# Autodesk Inventor assembly: robot
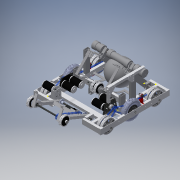
[picture p0: Inventor's stored thumbnail of the model, 180x180]
Saved by Autodesk Inventor 2016 (Build 200138000, 138)
## iProperties
Created: 2016-01-18
Part Number: robot
Document SubType Name: Assembly
Designer: gus
Mass: 30875.5 g
Surface Area: 55089.9 cm^2
Volume: 19218.2 cm^3
Density: 1.60657 g/cm^3
Author: gus
## Documents named in this file (36)
- \\Mac\Home\Desktop\1510-stronghold-CAD-master\robot.iam
- \\Mac\Home\Desktop\1510-stronghold-CAD-master\chassis\chassis.iam
- \\Mac\Home\Desktop\1510-stronghold-CAD-master\roller wheels\roller wheels.iam
- \\Mac\Home\Desktop\1510-stronghold-CAD-master\chassis\chain tensioner\chain tensioner.iam
- \\Mac\Home\Desktop\1510-stronghold-CAD-master\pickeruperthingy\armAssembaly.iam
- \\Mac\Home\Desktop\1510-stronghold-CAD-master\pickeruperthingy\2x2block.ipt
- \\Mac\Home\Desktop\1510-stronghold-CAD-master\pickeruperthingy\Roller Drum 10-Inch.ipt
- \\Mac\Home\Desktop\1510-stronghold-CAD-master\pickeruperthingy\Roller Drum 4-Inch.ipt
- \\Mac\Home\Desktop\1510-stronghold-CAD-master\roller wheels\4-in higrip\4 in HiGrip Wheel.iam
- \\Mac\Home\Desktop\1510-stronghold-CAD-master\pickeruperthingy\Part13.ipt
- \\Mac\Home\Desktop\1510-stronghold-CAD-master\shooter\Part4.ipt
- \\Mac\Home\Desktop\1510-stronghold-CAD-master\shooter\railtop.ipt
- \\Mac\Home\Desktop\1510-stronghold-CAD-master\shooter\superstructure.ipt
- \\Mac\Home\Desktop\1510-stronghold-CAD-master\shooter\supportbeam1.ipt
- \\Mac\Home\Desktop\1510-stronghold-CAD-master\shooter\supportblock1.ipt
- \\Mac\Home\Desktop\1510-stronghold-CAD-master\shooter\supportbeam2.ipt
- \\Mac\Home\Desktop\1510-stronghold-CAD-master\shooter\superstructure2.ipt
- \\Mac\Home\Desktop\1510-stronghold-CAD-master\shooter\flywheelsupport.ipt
- \\Mac\Home\Desktop\1510-stronghold-CAD-master\shooter\flywheelsupport2.ipt
- \\Mac\Home\Desktop\1510-stronghold-CAD-master\shooter\aimingrails.ipt
- \\Mac\Home\Desktop\1510-stronghold-CAD-master\shooter\bolt.ipt
- \\Mac\Home\Desktop\1510-stronghold-CAD-master\shooter\boltholder.ipt
- \\Mac\Home\Desktop\1510-stronghold-CAD-master\shooter\aimingcontrol.ipt
- \\Mac\Home\Desktop\1510-stronghold-CAD-master\pickeruperthingy\rollerwheelpoweraxel.ipt
- \\Mac\Home\Desktop\1510-stronghold-CAD-master\pickeruperthingy\217-3875-STEP-20140818.ipt
- \\Mac\Home\Desktop\1510-stronghold-CAD-master\roller wheels\am-0096a+500+Hex+Hub+r2.ipt
- \\Mac\Home\Desktop\1510-stronghold-CAD-master\pickeruperthingy\rod3.ipt
- \\Mac\Home\Desktop\1510-stronghold-CAD-master\pickeruperthingy\217-2704.20121204.ipt
- \\Mac\Home\Desktop\1510-stronghold-CAD-master\roller cage\roller cage.iam
- \\Mac\Home\Desktop\1510-stronghold-CAD-master\ball.ipt
- \\Mac\Home\Desktop\1510-stronghold-CAD-master\shooter\am-2231a+375+Hex+Hub+r3.ipt
- \\Mac\Home\Desktop\1510-stronghold-CAD-master\shooter\217-2735.20121205-2.ipt
- \\Mac\Home\Desktop\1510-stronghold-CAD-master\roller cage\3-8 hex axle.ipt
- \\Mac\Home\Desktop\1510-stronghold-CAD-master\shooter\fly wheel gusset.ipt
- \\Mac\Home\Desktop\1510-stronghold-CAD-master\shooter\angle gusset.ipt
- \\Mac\Home\Desktop\1510-stronghold-CAD-master\shooter\angle gusset 2.ipt
## Components (72 placed, 35 different names)
1. chassis:1 [sub-assembly] — Cylindrical:1, Mate:1, Flush:1, Mate:3, Flush:2, Mate:4, Mate:5, Flush:3, Flush:4, Flush:5, Flush:6, Mate:6, Mate:16, Flush:22, Mate:23, Flush:23, Flush:24, Mate:24, Mate:25, Mate:35, Mate:37, Mate:40, Mate:41, Flush:37, Mate:43, Flush:41, Mate:107, Mate:115, Flush:81, Flush:82, Mate:116, Flush:83, Mate:119
2. roller wheels:1 [sub-assembly] — Cylindrical:1, Mate:1
3. chain tensioner:1 [sub-assembly] — Flush:1
4. chain tensioner:2 [sub-assembly] — Mate:3, Flush:2
5. armAssembaly:1 [sub-assembly] — Mate:4, Mate:7, Mate:8, Mate:9, Mate:10, Mate:11, Mate:12, Flush:7, Mate:13, Mate:14, Flush:8, Flush:12, Flush:74, Mate:78, Mate:79, Mate:80, Mate:81
6. 2x2block:1 — Mate:5, Flush:3, Flush:4, Mate:76, Mate:77
7. 2x2block:2 — Flush:5, Flush:6, Mate:6, Mate:7, Mate:72, Mate:73
8. Roller Drum 10-Inch:1 — Mate:8, Mate:9, Mate:10, Mate:78
9. Roller Drum 4-Inch:1 — Mate:13, Mate:14, Flush:8
10. Roller Drum 4-Inch:2 — Mate:11, Mate:12, Flush:7
11. 4 in HiGrip Wheel:1 [sub-assembly] — Mate:47, Mate:88, Mate:89, Mate:90, Mate:91, Mate:92, Mate:93, Mate:107
12. Part13:1 — Mate:16, Flush:12, Mate:17, Flush:13, Flush:14, Mate:18, Flush:15, Mate:19, Mate:33, Flush:32, Mate:34
13. Part13:2 — Mate:17, Flush:13, Flush:14, Mate:25, Flush:33, Mate:36
14. Part4:1 — Mate:18, Flush:15, Mate:19, Mate:20, Flush:16, Flush:17, Flush:35, Flush:36, Mate:38, Flush:62, Mate:58, Flush:63, Flush:64
15. Part4:2 — Mate:20, Flush:16, Flush:17, Flush:18, Flush:19, Mate:21, Flush:39, Flush:40, Flush:58, Flush:59, Flush:60, Mate:56, Flush:61, Flush:66
16. railtop:1 — Flush:18, Flush:19, Mate:21, Mate:22, Flush:20, Flush:21, Flush:26, Flush:27, Flush:48, Flush:50
17. railtop:2 — Mate:22, Flush:20, Flush:21, Flush:29, Flush:30, Mate:53, Flush:53, Flush:54, Flush:55
18. superstructure:1 — Flush:22, Mate:23, Flush:23, Flush:25, Mate:29, Mate:31, Flush:34, Mate:39, Mate:40, Mate:87, Flush:76
19. superstructure:2 — Flush:24, Mate:24, Flush:25, Mate:26, Mate:28
20. supportbeam1:1 — Mate:26, Flush:26, Flush:27, Mate:27, Flush:28, Mate:49, Flush:51
21. supportblock1:1 — Mate:27, Flush:28, Mate:28
22. supportbeam2:1 — Mate:29, Flush:29, Flush:30, Flush:31, Mate:30, Flush:57
23. supportblock1:2 — Flush:31, Mate:30, Mate:31
24. supportbeam2:2 — Mate:33, Flush:32, Mate:34
25. supportbeam1:2 — Mate:35, Flush:33, Mate:36
26. superstructure2:1 — Mate:37, Flush:34, Mate:39, Flush:38
27. supportbeam2:3 — Flush:35, Flush:36, Mate:38
28. superstructure2:2 — Mate:41, Flush:37, Flush:38, Mate:42
29. supportbeam1:3 — Flush:39, Flush:40, Mate:42
30. flywheelsupport:1 — Mate:43, Flush:41, Flush:42, Flush:43, Flush:46, Mate:48, Flush:47, Mate:112, Mate:117, Mate:118
31. flywheelsupport:2 — Flush:42, Flush:43, Mate:46, Flush:44, Flush:45, Mate:110, Mate:114
32. flywheelsupport2:1 — Mate:46, Flush:44, Flush:45, Mate:47, Mate:101, Mate:102, Mate:103, Mate:104, Mate:111, Flush:79
33. flywheelsupport2:2 — Flush:46, Mate:48, Flush:47, Mate:97, Mate:98, Mate:99, Mate:100, Flush:80, Mate:113
34. aimingrails:1 — Mate:51, Mate:52, Mate:63, Mate:65, Flush:69
35. bolt:1 — Mate:50, Mate:51, Mate:52, Flush:50
36. boltholder:1 — Mate:49, Flush:48, Mate:50, Flush:51
37. boltholder:2 — Mate:53, Flush:53, Mate:54, Flush:57
38. bolt:2 — Mate:54, Flush:54, Mate:55
39. aimingrails:2 — Mate:55, Flush:55, Mate:63, Mate:67, Flush:71
40. boltholder:3 — Flush:58, Flush:59, Flush:60, Mate:56, Mate:57
41. bolt:3 — Mate:57, Flush:61, Mate:61
42. boltholder:4 — Flush:62, Mate:58, Flush:63, Mate:59
43. bolt:4 — Mate:59, Flush:64, Mate:60, Flush:65
44. aimingrails:3 — Mate:60, Flush:65, Mate:62, Mate:66, Flush:70
45. aimingrails:4 — Mate:61, Flush:66, Mate:62, Mate:64, Flush:68
46. bolt:5 — Mate:64, Flush:68, Mate:70
47. bolt:6 — Mate:65, Flush:69, Mate:71, Flush:73
48. bolt:7 — Mate:66, Flush:70, Mate:69, Flush:72
49. bolt:8 — Mate:67, Flush:71, Mate:68
50. aimingcontrol:1 — Mate:68, Mate:69, Flush:72
51. aimingcontrol:2 — Mate:70, Mate:71, Flush:73
52. rollerwheelpoweraxel:1 — Mate:74, Mate:75, Flush:74
53. 217-3875-STEP-20140818:1 — Mate:72, Mate:73, Mate:74, Mate:75
54. 217-3875-STEP-20140818:2 — Mate:76, Mate:77, Mate:86
55. am-0096a+500+Hex+Hub+r2:1 — Mate:79, Flush:75, Mate:82, Mate:83
56. rod3:1 — Mate:80, Mate:81, Flush:75, Mate:82, Mate:83, Mate:84, Mate:85
57. 217-2704.20121204:1 — Mate:84, Mate:85, Mate:86
58. roller cage:1 [sub-assembly] — Mate:87, Flush:76
59. ball:1
60. 4 in HiGrip Wheel:2 [sub-assembly] — Mate:88, Mate:89, Mate:90, Mate:94, Mate:95, Mate:96
61. am-2231a+375+Hex+Hub+r3:1 — Mate:91, Mate:92, Mate:93, Mate:106
62. am-2231a+375+Hex+Hub+r3:2 — Mate:94, Mate:95, Mate:96, Mate:105
63. 217-2735.20121205-2:1 — Mate:101, Mate:102, Flush:78
64. 217-2735.20121205-2:2 — Mate:98, Flush:77, Mate:99, Mate:105, Mate:108, Mate:109
65. 217-2735.20121205-2:3 — Mate:103, Mate:104, Flush:78, Mate:106
66. 217-2735.20121205-2:4 — Mate:97, Flush:77, Mate:100
67. 3-8 hex axle:1 — Mate:108, Mate:109
68. fly wheel gusset:1 — Mate:110, Mate:111, Flush:79
69. fly wheel gusset:2 — Flush:80, Mate:112, Mate:113
70. angle gusset:1 — Mate:114, Mate:115, Flush:81
71. angle gusset:2 — Flush:82, Mate:116, Mate:117
72. angle gusset 2:1 — Mate:118, Flush:83, Mate:119
## Relationships (191: Mate 114, Flush 76, CylindricalJoint 1)
- Cylindrical:1: chassis:1 ↔ roller wheels:1
- Mate:1 (10.16 mm): chassis:1 ↔ roller wheels:1
- Flush:1: chassis:1 ↔ chain tensioner:1
- Mate:3: chassis:1 ↔ chain tensioner:2
- Flush:2: chassis:1 ↔ chain tensioner:2
- Mate:4: chassis:1 ↔ armAssembaly:1
- Mate:5: chassis:1 ↔ 2x2block:1
- Flush:3: chassis:1 ↔ 2x2block:1
- Flush:4: chassis:1 ↔ 2x2block:1
- Flush:5: chassis:1 ↔ 2x2block:2
- Flush:6: chassis:1 ↔ 2x2block:2
- Mate:6: chassis:1 ↔ 2x2block:2
- Mate:7: armAssembaly:1 ↔ 2x2block:2
- Mate:8: armAssembaly:1 ↔ Roller Drum 10-Inch:1
- Mate:9: armAssembaly:1 ↔ Roller Drum 10-Inch:1
- Mate:10 (25.4 mm): armAssembaly:1 ↔ Roller Drum 10-Inch:1
- Mate:11: armAssembaly:1 ↔ Roller Drum 4-Inch:2
- Mate:12: armAssembaly:1 ↔ Roller Drum 4-Inch:2
- Flush:7: armAssembaly:1 ↔ Roller Drum 4-Inch:2
- Mate:13: armAssembaly:1 ↔ Roller Drum 4-Inch:1
- Mate:14: armAssembaly:1 ↔ Roller Drum 4-Inch:1
- Flush:8: armAssembaly:1 ↔ Roller Drum 4-Inch:1
- Mate:16 (190.5 mm): chassis:1 ↔ Part13:1
- Flush:12: armAssembaly:1 ↔ Part13:1
- Mate:17 (190.5 mm): Part13:1 ↔ Part13:2
- Flush:13: Part13:1 ↔ Part13:2
- Flush:14: Part13:1 ↔ Part13:2
- Mate:18: Part13:1 ↔ Part4:1
- Flush:15: Part13:1 ↔ Part4:1
- Mate:19: Part13:1 ↔ Part4:1
- Mate:20 (190.5 mm): Part4:1 ↔ Part4:2
- Flush:16: Part4:1 ↔ Part4:2
- Flush:17: Part4:1 ↔ Part4:2
- Flush:18: Part4:2 ↔ railtop:1
- Flush:19: Part4:2 ↔ railtop:1
- Mate:21 (190.5 mm): Part4:2 ↔ railtop:1
- Mate:22 (190.5 mm): railtop:1 ↔ railtop:2
- Flush:20: railtop:1 ↔ railtop:2
- Flush:21: railtop:1 ↔ railtop:2
- Flush:22: chassis:1 ↔ superstructure:1
- Mate:23: chassis:1 ↔ superstructure:1
- Flush:23: chassis:1 ↔ superstructure:1
- Flush:24: chassis:1 ↔ superstructure:2
- Mate:24: chassis:1 ↔ superstructure:2
- Flush:25: superstructure:1 ↔ superstructure:2
- Mate:25 (-23.8125 mm): chassis:1 ↔ Part13:2
- Mate:26: superstructure:2 ↔ supportbeam1:1
- Flush:26: railtop:1 ↔ supportbeam1:1
- Flush:27: railtop:1 ↔ supportbeam1:1
- Mate:27: supportbeam1:1 ↔ supportblock1:1
- Flush:28: supportbeam1:1 ↔ supportblock1:1
- Mate:28: superstructure:2 ↔ supportblock1:1
- Mate:29: superstructure:1 ↔ supportbeam2:1
- Flush:29: railtop:2 ↔ supportbeam2:1
- Flush:30: railtop:2 ↔ supportbeam2:1
- Flush:31: supportbeam2:1 ↔ supportblock1:2
- Mate:30: supportbeam2:1 ↔ supportblock1:2
- Mate:31: superstructure:1 ↔ supportblock1:2
- Mate:33: Part13:1 ↔ supportbeam2:2
- Flush:32: Part13:1 ↔ supportbeam2:2
- Mate:34: Part13:1 ↔ supportbeam2:2
- Mate:35: chassis:1 ↔ supportbeam1:2
- Flush:33: Part13:2 ↔ supportbeam1:2
- Mate:36: Part13:2 ↔ supportbeam1:2
- Mate:37: chassis:1 ↔ superstructure2:1
- Flush:34: superstructure:1 ↔ superstructure2:1
- Flush:35: Part4:1 ↔ supportbeam2:3
- Flush:36: Part4:1 ↔ supportbeam2:3
- Mate:38: Part4:1 ↔ supportbeam2:3
- Mate:39 (63.5 mm): superstructure:1 ↔ superstructure2:1
- Mate:40 (12.7 mm): chassis:1 ↔ superstructure:1
- Mate:41: chassis:1 ↔ superstructure2:2
- Flush:37: chassis:1 ↔ superstructure2:2
- Flush:38: superstructure2:1 ↔ superstructure2:2
- Flush:39: Part4:2 ↔ supportbeam1:3
- Flush:40: Part4:2 ↔ supportbeam1:3
- Mate:42: superstructure2:2 ↔ supportbeam1:3
- Mate:43: chassis:1 ↔ flywheelsupport:1
- Flush:41: chassis:1 ↔ flywheelsupport:1
- Flush:42: flywheelsupport:1 ↔ flywheelsupport:2
- Flush:43: flywheelsupport:1 ↔ flywheelsupport:2
- Mate:46: flywheelsupport:2 ↔ flywheelsupport2:1
- Flush:44: flywheelsupport:2 ↔ flywheelsupport2:1
- Flush:45: flywheelsupport:2 ↔ flywheelsupport2:1
- Mate:47: 4 in HiGrip Wheel:1 ↔ flywheelsupport2:1
- Flush:46: flywheelsupport:1 ↔ flywheelsupport2:2
- Mate:48: flywheelsupport:1 ↔ flywheelsupport2:2
- Flush:47: flywheelsupport:1 ↔ flywheelsupport2:2
- Mate:49: supportbeam1:1 ↔ boltholder:1
- Flush:48 (25.4 mm): railtop:1 ↔ boltholder:1
- Mate:50: bolt:1 ↔ boltholder:1
- Mate:51: aimingrails:1 ↔ bolt:1
- Mate:52: aimingrails:1 ↔ bolt:1
- Flush:50: railtop:1 ↔ bolt:1
- Flush:51: supportbeam1:1 ↔ boltholder:1
- Mate:53: railtop:2 ↔ boltholder:2
- Flush:53 (25.4 mm): railtop:2 ↔ boltholder:2
- Mate:54: boltholder:2 ↔ bolt:2
- Flush:54: railtop:2 ↔ bolt:2
- Mate:55: bolt:2 ↔ aimingrails:2
- Flush:55: railtop:2 ↔ aimingrails:2
- Flush:57: supportbeam2:1 ↔ boltholder:2
- Flush:58: Part4:2 ↔ boltholder:3
- Flush:59 (25.4 mm): Part4:2 ↔ boltholder:3
- Flush:60: Part4:2 ↔ boltholder:3
- Mate:56: Part4:2 ↔ boltholder:3
- Mate:57: boltholder:3 ↔ bolt:3
- Flush:61: Part4:2 ↔ bolt:3
- Flush:62: Part4:1 ↔ boltholder:4
- Mate:58: Part4:1 ↔ boltholder:4
- Flush:63 (25.4 mm): Part4:1 ↔ boltholder:4
- Mate:59: boltholder:4 ↔ bolt:4
- Flush:64: Part4:1 ↔ bolt:4
- Mate:60: bolt:4 ↔ aimingrails:3
- Flush:65: bolt:4 ↔ aimingrails:3
- Mate:61: bolt:3 ↔ aimingrails:4
- Flush:66: Part4:2 ↔ aimingrails:4
- Mate:62: aimingrails:3 ↔ aimingrails:4
- Mate:63: aimingrails:1 ↔ aimingrails:2
- Mate:64: aimingrails:4 ↔ bolt:5
- Flush:68: aimingrails:4 ↔ bolt:5
- Mate:65: aimingrails:1 ↔ bolt:6
- Flush:69: aimingrails:1 ↔ bolt:6
- Mate:66: aimingrails:3 ↔ bolt:7
- Mate:67: aimingrails:2 ↔ bolt:8
- Flush:70: aimingrails:3 ↔ bolt:7
- Flush:71: aimingrails:2 ↔ bolt:8
- Mate:68: bolt:8 ↔ aimingcontrol:1
- Mate:69: bolt:7 ↔ aimingcontrol:1
- Flush:72: bolt:7 ↔ aimingcontrol:1
- Mate:70: bolt:5 ↔ aimingcontrol:2
- Mate:71: bolt:6 ↔ aimingcontrol:2
- Flush:73: bolt:6 ↔ aimingcontrol:2
- Mate:72: 2x2block:2 ↔ 217-3875-STEP-20140818:1
- Mate:73: 2x2block:2 ↔ 217-3875-STEP-20140818:1
- Mate:74: rollerwheelpoweraxel:1 ↔ 217-3875-STEP-20140818:1
- Mate:75: rollerwheelpoweraxel:1 ↔ 217-3875-STEP-20140818:1
- Flush:74: armAssembaly:1 ↔ rollerwheelpoweraxel:1
- Mate:76: 2x2block:1 ↔ 217-3875-STEP-20140818:2
- Mate:77: 2x2block:1 ↔ 217-3875-STEP-20140818:2
- Mate:78 (25.4 mm): armAssembaly:1 ↔ Roller Drum 10-Inch:1
- Mate:79: armAssembaly:1 ↔ am-0096a+500+Hex+Hub+r2:1
- Mate:80: armAssembaly:1 ↔ rod3:1
- Mate:81: armAssembaly:1 ↔ rod3:1
- Flush:75: am-0096a+500+Hex+Hub+r2:1 ↔ rod3:1
- Mate:82: am-0096a+500+Hex+Hub+r2:1 ↔ rod3:1
- Mate:83: am-0096a+500+Hex+Hub+r2:1 ↔ rod3:1
- Mate:84: rod3:1 ↔ 217-2704.20121204:1
- Mate:85: rod3:1 ↔ 217-2704.20121204:1
- Mate:86: 217-3875-STEP-20140818:2 ↔ 217-2704.20121204:1
- Mate:87: superstructure:1 ↔ roller cage:1
- Flush:76: superstructure:1 ↔ roller cage:1
- Mate:88: 4 in HiGrip Wheel:1 ↔ 4 in HiGrip Wheel:2
- Mate:89: 4 in HiGrip Wheel:1 ↔ 4 in HiGrip Wheel:2
- Mate:90: 4 in HiGrip Wheel:1 ↔ 4 in HiGrip Wheel:2
- Mate:91: 4 in HiGrip Wheel:1 ↔ am-2231a+375+Hex+Hub+r3:1
- Mate:92: 4 in HiGrip Wheel:1 ↔ am-2231a+375+Hex+Hub+r3:1
- Mate:93: 4 in HiGrip Wheel:1 ↔ am-2231a+375+Hex+Hub+r3:1
- Mate:94: 4 in HiGrip Wheel:2 ↔ am-2231a+375+Hex+Hub+r3:2
- Mate:95: 4 in HiGrip Wheel:2 ↔ am-2231a+375+Hex+Hub+r3:2
- Mate:96: 4 in HiGrip Wheel:2 ↔ am-2231a+375+Hex+Hub+r3:2
- Mate:97: flywheelsupport2:2 ↔ 217-2735.20121205-2:4
- Mate:98: flywheelsupport2:2 ↔ 217-2735.20121205-2:2
- Flush:77: 217-2735.20121205-2:2 ↔ 217-2735.20121205-2:4
- Mate:99: flywheelsupport2:2 ↔ 217-2735.20121205-2:2
- Mate:100: flywheelsupport2:2 ↔ 217-2735.20121205-2:4
- Mate:101: flywheelsupport2:1 ↔ 217-2735.20121205-2:1
- Mate:102: flywheelsupport2:1 ↔ 217-2735.20121205-2:1
- Mate:103: flywheelsupport2:1 ↔ 217-2735.20121205-2:3
- Mate:104: flywheelsupport2:1 ↔ 217-2735.20121205-2:3
- Flush:78: 217-2735.20121205-2:1 ↔ 217-2735.20121205-2:3
- Mate:105: am-2231a+375+Hex+Hub+r3:2 ↔ 217-2735.20121205-2:2
- Mate:106: am-2231a+375+Hex+Hub+r3:1 ↔ 217-2735.20121205-2:3
- Mate:107 (241.3 mm): chassis:1 ↔ 4 in HiGrip Wheel:1
- Mate:108: 217-2735.20121205-2:2 ↔ 3-8 hex axle:1
- Mate:109: 217-2735.20121205-2:2 ↔ 3-8 hex axle:1
- Mate:110: flywheelsupport:2 ↔ fly wheel gusset:1
- Mate:111: flywheelsupport2:1 ↔ fly wheel gusset:1
- Flush:79: flywheelsupport2:1 ↔ fly wheel gusset:1
- Flush:80: flywheelsupport2:2 ↔ fly wheel gusset:2
- Mate:112: flywheelsupport:1 ↔ fly wheel gusset:2
- Mate:113: flywheelsupport2:2 ↔ fly wheel gusset:2
- Mate:114: flywheelsupport:2 ↔ angle gusset:1
- Mate:115: chassis:1 ↔ angle gusset:1
- Flush:81: chassis:1 ↔ angle gusset:1
- Flush:82: chassis:1 ↔ angle gusset:2
- Mate:116: chassis:1 ↔ angle gusset:2
- Mate:117: flywheelsupport:1 ↔ angle gusset:2
- Mate:118: flywheelsupport:1 ↔ angle gusset 2:1
- Flush:83: chassis:1 ↔ angle gusset 2:1
- Mate:119: chassis:1 ↔ angle gusset 2:1
